# Autodesk Inventor assembly: SFU1605-3_MIR
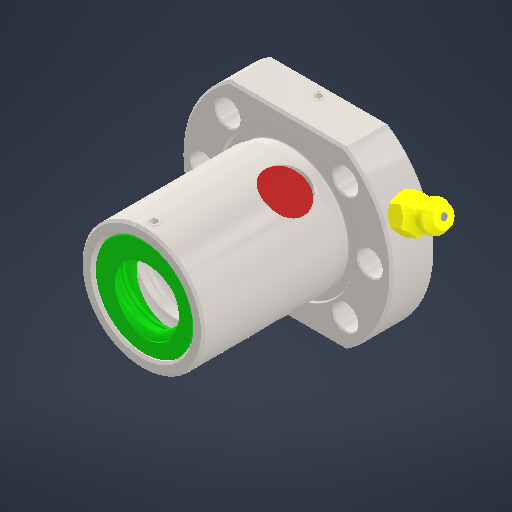
[picture p0: Inventor's stored thumbnail of the model, 512x512]
Saved by Autodesk Inventor 2026.2 (Build 302298000, 298)
## iProperties
Created: 2026-06-14
Part Number: SFU1605-3_MIR
Description: STEP AP214
Document SubType Name: Assembly
Designer: Kenji
Sending System: Autodesk Inventor 2026
Preprocessor: ST-DEVELOPER v20.1
Title: SFU1605-3_MIR.stp
Author: Kenji
Revision Number: ANY
## Documents named in this file (7)
- C:\Users\Kenji\Documents\GitHub\DiyCNC-\COTS-Parts\SFU1605-BallScrewNut.iam
- C:\Users\Kenji\Downloads\SFU1605-3_MIR\SFU1605-3_MIR\SFU Ball Nut_1605-3_MIR.ipt
- C:\Users\Kenji\Downloads\SFU1605-3_MIR\SFU1605-3_MIR\SFU1605 Washer Front_MIR.ipt
- C:\Users\Kenji\Downloads\SFU1605-3_MIR\SFU1605-3_MIR\SFU1605 Washer Back_MIR.ipt
- C:\Users\Kenji\Downloads\SFU1605-3_MIR\SFU1605-3_MIR\Grease Nipple A M6x1.00_MIR.iam
- C:\Users\Kenji\Downloads\SFU1605-3_MIR\SFU1605-3_MIR\socket set screw cone point_iso_ISO 4027 - M3 x 5-C_MIR.ipt
- C:\Users\Kenji\Downloads\SFU1605-3_MIR\SFU1605-3_MIR\socket set screw cone point_iso_ISO 4027 - M3 x 2.5-C_MIR.ipt
## Components (8 placed, 6 different names)
1. SFU Ball Nut_1605-3_MIR:1 — Mate:1, Mate:2, Mate:3, Mate:4, Mate:5, Tangent:1, Mate:6, Tangent:2, Mate:7, Flush:1, Mate:8, Flush:2, Mate:9, Tangent:3
2. SFU1605 Washer Front_MIR:1 — Mate:1, Mate:2
3. SFU1605 Washer Back_MIR:1 — Mate:3, Mate:4
4. Grease Nipple A M6x1.00_MIR:1 [sub-assembly] — Mate:9, Tangent:3
5. socket set screw cone point_iso_ISO 4027 - M3 x 5-C_MIR:1 — Mate:7, Flush:1
6. socket set screw cone point_iso_ISO 4027 - M3 x 5-C_MIR:2 — Mate:8, Flush:2
7. socket set screw cone point_iso_ISO 4027 - M3 x 2.5-C_MIR:1 — Mate:6, Tangent:2
8. socket set screw cone point_iso_ISO 4027 - M3 x 2.5-C_MIR:2 — Mate:5, Tangent:1
## Relationships (14: Mate 9, Tangent 3, Flush 2)
- Mate:1: SFU Ball Nut_1605-3_MIR:1 ↔ SFU1605 Washer Front_MIR:1
- Mate:2: SFU Ball Nut_1605-3_MIR:1 ↔ SFU1605 Washer Front_MIR:1
- Mate:3: SFU Ball Nut_1605-3_MIR:1 ↔ SFU1605 Washer Back_MIR:1
- Mate:4: SFU Ball Nut_1605-3_MIR:1 ↔ SFU1605 Washer Back_MIR:1
- Mate:5: SFU Ball Nut_1605-3_MIR:1 ↔ socket set screw cone point_iso_ISO 4027 - M3 x 2.5-C_MIR:2
- Tangent:1: SFU Ball Nut_1605-3_MIR:1 ↔ socket set screw cone point_iso_ISO 4027 - M3 x 2.5-C_MIR:2
- Mate:6: SFU Ball Nut_1605-3_MIR:1 ↔ socket set screw cone point_iso_ISO 4027 - M3 x 2.5-C_MIR:1
- Tangent:2: SFU Ball Nut_1605-3_MIR:1 ↔ socket set screw cone point_iso_ISO 4027 - M3 x 2.5-C_MIR:1
- Mate:7: SFU Ball Nut_1605-3_MIR:1 ↔ socket set screw cone point_iso_ISO 4027 - M3 x 5-C_MIR:1
- Flush:1: SFU Ball Nut_1605-3_MIR:1 ↔ socket set screw cone point_iso_ISO 4027 - M3 x 5-C_MIR:1
- Mate:8: SFU Ball Nut_1605-3_MIR:1 ↔ socket set screw cone point_iso_ISO 4027 - M3 x 5-C_MIR:2
- Flush:2: SFU Ball Nut_1605-3_MIR:1 ↔ socket set screw cone point_iso_ISO 4027 - M3 x 5-C_MIR:2
- Mate:9: SFU Ball Nut_1605-3_MIR:1 ↔ Grease Nipple A M6x1.00_MIR:1
- Tangent:3: SFU Ball Nut_1605-3_MIR:1 ↔ Grease Nipple A M6x1.00_MIR:1
